# Autodesk Inventor assembly: turtlebot_installation
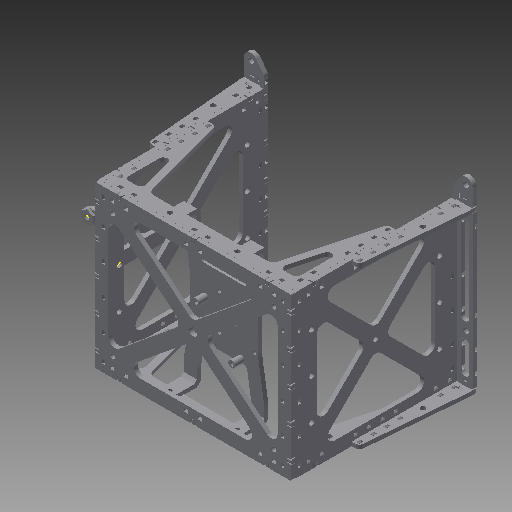
[picture p0: Inventor's stored thumbnail of the model, 512x512]
Saved by Autodesk Inventor 2018 (Build 220112000, 112)
## iProperties
Created: 2018-07-15
Part Number: turtlebot_installation
Document SubType Name: Assembly
Designer: Tsche
Author: Tsche
## Documents named in this file (9)
- C:\Users\Tsche\Documents\MSE\MA\turtlebot_mods\turtlebot_installation.iam
- C:\Users\Tsche\Documents\MSE\MA\turtlebot_mods\turtlebot_installation_bottom_left.ipt
- C:\Users\Tsche\Documents\MSE\MA\turtlebot_mods\turtlebot_installation_side.ipt
- C:\Users\Tsche\Documents\MSE\MA\turtlebot_mods\turtlebot_installation_fin_bottom.ipt
- C:\Users\Tsche\Documents\MSE\MA\turtlebot_mods\turtlebot_installation_top.ipt
- C:\Users\Tsche\Documents\MSE\MA\turtlebot_mods\turtlebot_installation_fin_top.ipt
- C:\Users\Tsche\Documents\MSE\MA\turtlebot_mods\turtlebot_installation_bottom_right.ipt
- C:\Users\Tsche\Documents\MSE\MA\turtlebot_mods\GPS_holder.ipt
- C:\Users\Tsche\Documents\MSE\MA\turtlebot_mods\IMU_holder.ipt
## Components (13 placed, 8 different names)
1. turtlebot_installation_bottom_left:1 — Flush:2, Mate:1, Mate:3, Mate:4, Flush:5, Mate:15, Flush:20
2. turtlebot_installation_side:1 — Flush:2, Mate:1, Mate:5, Mate:7, Flush:3, Flush:4, Flush:5, Mate:8, Flush:6, Flush:7, Mate:9, Flush:8, Flush:9, Mate:10, Flush:10, Flush:11, Mate:16, Mate:17, Mate:18
3. turtlebot_installation_fin_bottom:1 — Mate:3, Mate:7, Flush:3
4. turtlebot_installation_fin_bottom:2 — Mate:4, Mate:5, Flush:4
5. turtlebot_installation_fin_top:1 — Mate:9, Flush:8, Flush:9, Mate:11, Flush:12, Flush:13
6. turtlebot_installation_fin_top:2 — Mate:10, Flush:10, Flush:11, Mate:19, Mate:20, Mate:21
7. turtlebot_installation_top:1 — Mate:8, Flush:6, Flush:7, Flush:21
8. turtlebot_installation_side:2 — Mate:11, Flush:12, Flush:13, Mate:12, Flush:14, Flush:15, Mate:13, Flush:16, Flush:17, Mate:14, Flush:18, Flush:19
9. turtlebot_installation_fin_bottom:3 — Mate:12, Flush:14, Flush:15
10. turtlebot_installation_fin_bottom:4 — Mate:13, Flush:16, Flush:17
11. turtlebot_installation_bottom_right:1 — Mate:14, Flush:18, Flush:19
12. GPS_holder:1 — Mate:16, Mate:17, Mate:18
13. IMU_holder:1 — Mate:19, Mate:20, Mate:21
## Relationships (39: Flush 20, Mate 19)
- Flush:2: turtlebot_installation_bottom_left:1 ↔ turtlebot_installation_side:1
- Mate:1: turtlebot_installation_bottom_left:1 ↔ turtlebot_installation_side:1
- Mate:3: turtlebot_installation_bottom_left:1 ↔ turtlebot_installation_fin_bottom:1
- Mate:4: turtlebot_installation_bottom_left:1 ↔ turtlebot_installation_fin_bottom:2
- Mate:5: turtlebot_installation_side:1 ↔ turtlebot_installation_fin_bottom:2
- Mate:7: turtlebot_installation_side:1 ↔ turtlebot_installation_fin_bottom:1
- Flush:3: turtlebot_installation_side:1 ↔ turtlebot_installation_fin_bottom:1
- Flush:4: turtlebot_installation_side:1 ↔ turtlebot_installation_fin_bottom:2
- Flush:5: turtlebot_installation_bottom_left:1 ↔ turtlebot_installation_side:1
- Mate:8: turtlebot_installation_side:1 ↔ turtlebot_installation_top:1
- Flush:6: turtlebot_installation_side:1 ↔ turtlebot_installation_top:1
- Flush:7: turtlebot_installation_side:1 ↔ turtlebot_installation_top:1
- Mate:9: turtlebot_installation_side:1 ↔ turtlebot_installation_fin_top:1
- Flush:8: turtlebot_installation_side:1 ↔ turtlebot_installation_fin_top:1
- Flush:9: turtlebot_installation_side:1 ↔ turtlebot_installation_fin_top:1
- Mate:10: turtlebot_installation_side:1 ↔ turtlebot_installation_fin_top:2
- Flush:10: turtlebot_installation_side:1 ↔ turtlebot_installation_fin_top:2
- Flush:11: turtlebot_installation_side:1 ↔ turtlebot_installation_fin_top:2
- Mate:11: turtlebot_installation_fin_top:1 ↔ turtlebot_installation_side:2
- Flush:12: turtlebot_installation_fin_top:1 ↔ turtlebot_installation_side:2
- Flush:13: turtlebot_installation_fin_top:1 ↔ turtlebot_installation_side:2
- Mate:12: turtlebot_installation_side:2 ↔ turtlebot_installation_fin_bottom:3
- Flush:14: turtlebot_installation_side:2 ↔ turtlebot_installation_fin_bottom:3
- Flush:15: turtlebot_installation_side:2 ↔ turtlebot_installation_fin_bottom:3
- Mate:13: turtlebot_installation_side:2 ↔ turtlebot_installation_fin_bottom:4
- Flush:16: turtlebot_installation_side:2 ↔ turtlebot_installation_fin_bottom:4
- Flush:17: turtlebot_installation_side:2 ↔ turtlebot_installation_fin_bottom:4
- Mate:14: turtlebot_installation_side:2 ↔ turtlebot_installation_bottom_right:1
- Flush:18: turtlebot_installation_side:2 ↔ turtlebot_installation_bottom_right:1
- Flush:19: turtlebot_installation_side:2 ↔ turtlebot_installation_bottom_right:1
- Mate:15: turtlebot_installation_bottom_left:1
- Flush:20: turtlebot_installation_bottom_left:1
- Flush:21: turtlebot_installation_top:1
- Mate:16: turtlebot_installation_side:1 ↔ GPS_holder:1
- Mate:17: turtlebot_installation_side:1 ↔ GPS_holder:1
- Mate:18: turtlebot_installation_side:1 ↔ GPS_holder:1
- Mate:19 (-0.5 mm): turtlebot_installation_fin_top:2 ↔ IMU_holder:1
- Mate:20: turtlebot_installation_fin_top:2 ↔ IMU_holder:1
- Mate:21: turtlebot_installation_fin_top:2 ↔ IMU_holder:1
